# Autodesk Inventor assembly: pcb
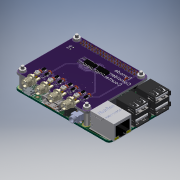
[picture p0: Inventor's stored thumbnail of the model, 180x180]
Saved by Autodesk Inventor 2016 (Build 200138000, 138)
## iProperties
Created: 2016-06-24
Part Number: pcb
Document SubType Name: Assembly
Designer: Jonathan
Author: Jonathan
## Documents named in this file (15)
- C:\Users\Jonathan\Documents\Projects\dynodePiShield\coincidenceCounter\cad\pcb.iam
- C:\Users\Jonathan\Documents\Projects\dynodePiShield\coincidenceCounter\cad\pcb.ipt
- C:\Users\Jonathan\Documents\Projects\dynodePiShield\coincidenceCounter\cad\electronics\SOT23-6.ipt
- C:\Users\Jonathan\Documents\Projects\dynodePiShield\coincidenceCounter\cad\electronics\resistor\chipResistor\chipResistor-0402.ipt
- C:\Users\Jonathan\Documents\Projects\dynodePiShield\coincidenceCounter\cad\electronics\resistor\chipResistor.ipt
- C:\Users\Jonathan\Documents\Projects\dynodePiShield\coincidenceCounter\cad\electronics\PVZ3A\PVZ3A.iam
- C:\Users\Jonathan\Documents\Projects\dynodePiShield\coincidenceCounter\cad\electronics\soic\soic-14-N.ipt
- C:\Users\Jonathan\Documents\Projects\dynodePiShield\coincidenceCounter\cad\electronics\soic\soic.ipt
- C:\Users\Jonathan\Documents\Projects\dynodePiShield\coincidenceCounter\cad\electronics\SMA Female Edge Mount CONSMA003-062.ipt
- C:\Users\Jonathan\Documents\Projects\dynodePiShield\coincidenceCounter\cad\wire.ipt
- C:\Users\Jonathan\Documents\Projects\dynodePiShield\coincidenceCounter\cad\electronics\femaleHeaders\femaleHeaders.iam
- C:\Users\Jonathan\Documents\Projects\dynodePiShield\coincidenceCounter\cad\electronics\raspberrypi_b_+_(assembly).ipt
- C:\Users\Jonathan\Documents\Projects\dynodePiShield\coincidenceCounter\cad\hardware\11mm M2.5 standoff.ipt
- C:\Users\Jonathan\Documents\Projects\dynodePiShield\coincidenceCounter\cad\hardware\M2.5 6mm screw.ipt
- C:\Users\Jonathan\Documents\Projects\dynodePiShield\coincidenceCounter\cad\hardware\M2.5 hex nut.ipt
## Components (54 placed, 12 different names)
1. pcb:1 — Mate:2, Angle:12, Mate:4, Angle:16, Mate:5, Mate:6, Mate:7, Mate:8, Mate:9, Mate:10, Angle:18, Angle:19, Angle:20, Angle:21, Angle:22, Angle:23, Angle:24, Angle:25, Mate:11, Mate:17, Mate:18, Mate:19, Mate:20, Flush:68, Flush:69, Mate:34, Mate:35, Mate:36, Mate:37
2. SOT23-6:1 — Flush:1, Flush:2, Flush:11, Mate:2
3. SOT23-6:2 — Flush:1, Flush:8
4. SOT23-6:3 — Flush:2, Flush:3, Flush:8, Flush:9
5. SOT23-6:4 — Flush:3, Flush:4, Flush:11, Flush:12
6. SOT23-6:5 — Flush:4, Flush:5, Flush:9, Flush:10
7. SOT23-6:6 — Flush:5, Flush:6, Flush:12, Flush:13
8. SOT23-6:7 — Flush:6, Flush:7, Flush:10
9. SOT23-6:8 — Flush:7, Flush:13
10. chipResistor-0402:3 — Flush:28, Flush:46, Mate:9
11. chipResistor-0402:4 — Flush:16, Flush:28, Flush:29, Flush:46
12. chipResistor-0402:7 — Flush:16, Flush:29, Flush:30, Flush:47
13. chipResistor-0402:10 — Flush:30, Flush:47
14. PVZ3A:1 [sub-assembly] — Angle:14, Angle:15, Flush:35, Flush:36, Flush:38, Flush:39, Mate:4
15. PVZ3A:2 [sub-assembly] — Angle:12, Angle:13, Flush:34, Flush:37
16. PVZ3A:3 [sub-assembly] — Angle:13, Angle:14, Flush:34, Flush:35, Flush:37, Flush:38
17. PVZ3A:4 [sub-assembly] — Angle:15, Flush:36, Flush:39
18. soic-14-N:1 — Angle:17, Mate:6
19. soic-14-N:2 — Angle:16, Angle:17, Mate:5
20. SMA Female Edge Mount CONSMA003-062:1 — Flush:42, Flush:45
21. SMA Female Edge Mount CONSMA003-062:2 — Flush:41, Flush:42, Flush:44, Flush:45
22. SMA Female Edge Mount CONSMA003-062:3 — Flush:40, Flush:41, Flush:43, Flush:44
23. SMA Female Edge Mount CONSMA003-062:4 — Flush:40, Flush:43, Mate:7, Mate:8
24. chipResistor-0402:11
25. chipResistor-0402:12
26. chipResistor-0402:13
27. chipResistor-0402:14
28. chipResistor-0402:15
29. chipResistor-0402:16
30. chipResistor-0402:17
31. chipResistor-0402:18
32. wire:1 — Flush:60, Flush:61, Angle:18
33. wire:2 — Flush:60, Flush:65, Mate:10, Angle:19
34. wire:3 — Flush:61, Flush:62, Angle:20
35. wire:4 — Flush:65, Flush:66, Angle:21
36. wire:5 — Flush:62, Flush:63, Angle:22
37. wire:6 — Flush:66, Flush:67, Angle:23
38. wire:7 — Flush:63, Flush:64, Angle:24
39. wire:8 — Flush:67, Angle:25
40. wire:9 — Flush:64
41. femaleHeaders:1 [sub-assembly] — Mate:11, Mate:12
42. raspberrypi_b_+_(assembly):1 — Mate:12, Mate:13, Mate:14, Mate:15, Mate:16, Angle:26, Angle:27, Mate:21, Mate:22, Mate:23, Mate:24, Flush:68, Flush:69, Mate:25, Mate:26, Mate:27, Mate:28
43. 11mm M2.5 standoff:1 — Mate:16, Mate:20, Angle:29, Angle:32, Mate:32, Angle:37
44. 11mm M2.5 standoff:2 — Mate:15, Mate:18, Angle:28, Angle:30, Mate:31, Angle:34
45. 11mm M2.5 standoff:3 — Mate:14, Mate:19, Angle:27, Angle:29, Mate:29, Angle:36
46. 11mm M2.5 standoff:4 — Mate:13, Mate:17, Angle:26, Angle:28, Angle:31, Mate:33, Angle:35
47. M2.5 6mm screw:1 — Mate:21, Mate:28, Angle:30
48. M2.5 6mm screw:2 — Mate:22, Mate:25, Angle:31
49. M2.5 6mm screw:3 — Mate:23, Mate:27, Angle:32, Angle:33
50. M2.5 6mm screw:4 — Mate:24, Mate:26, Angle:33
51. M2.5 hex nut:1 — Mate:33, Mate:34, Angle:35
52. M2.5 hex nut:2 — Mate:31, Mate:36, Angle:34
53. M2.5 hex nut:3 — Mate:32, Mate:37, Angle:37
54. M2.5 hex nut:4 — Mate:29, Mate:35, Angle:36
## Relationships (113: Flush 53, Mate 34, Angle 26)
- Flush:1: SOT23-6:1 ↔ SOT23-6:2
- Flush:2: SOT23-6:1 ↔ SOT23-6:3
- Flush:3: SOT23-6:3 ↔ SOT23-6:4
- Flush:4: SOT23-6:4 ↔ SOT23-6:5
- Flush:5: SOT23-6:5 ↔ SOT23-6:6
- Flush:6: SOT23-6:6 ↔ SOT23-6:7
- Flush:7: SOT23-6:7 ↔ SOT23-6:8
- Flush:8: SOT23-6:2 ↔ SOT23-6:3
- Flush:9: SOT23-6:3 ↔ SOT23-6:5
- Flush:10: SOT23-6:5 ↔ SOT23-6:7
- Flush:11: SOT23-6:1 ↔ SOT23-6:4
- Flush:12: SOT23-6:4 ↔ SOT23-6:6
- Flush:13: SOT23-6:6 ↔ SOT23-6:8
- Mate:2: pcb:1 ↔ SOT23-6:1
- Flush:16: chipResistor-0402:4 ↔ chipResistor-0402:7
- Flush:28: chipResistor-0402:3 ↔ chipResistor-0402:4
- Flush:29: chipResistor-0402:4 ↔ chipResistor-0402:7
- Flush:30: chipResistor-0402:7 ↔ chipResistor-0402:10
- Angle:12 (0 deg): pcb:1 ↔ PVZ3A:2
- Angle:13 (0 deg): PVZ3A:2 ↔ PVZ3A:3
- Angle:14 (0 deg): PVZ3A:1 ↔ PVZ3A:3
- Angle:15 (0 deg): PVZ3A:1 ↔ PVZ3A:4
- Flush:34: PVZ3A:2 ↔ PVZ3A:3
- Flush:35: PVZ3A:1 ↔ PVZ3A:3
- Flush:36: PVZ3A:1 ↔ PVZ3A:4
- Flush:37: PVZ3A:2 ↔ PVZ3A:3
- Flush:38: PVZ3A:1 ↔ PVZ3A:3
- Flush:39: PVZ3A:1 ↔ PVZ3A:4
- Mate:4: pcb:1 ↔ PVZ3A:1
- Angle:16 (0 deg): pcb:1 ↔ soic-14-N:2
- Angle:17 (0 deg): soic-14-N:1 ↔ soic-14-N:2
- Mate:5: pcb:1 ↔ soic-14-N:2
- Mate:6: pcb:1 ↔ soic-14-N:1
- Flush:40: SMA Female Edge Mount CONSMA003-062:3 ↔ SMA Female Edge Mount CONSMA003-062:4
- Flush:41: SMA Female Edge Mount CONSMA003-062:2 ↔ SMA Female Edge Mount CONSMA003-062:3
- Flush:42: SMA Female Edge Mount CONSMA003-062:1 ↔ SMA Female Edge Mount CONSMA003-062:2
- Flush:43: SMA Female Edge Mount CONSMA003-062:3 ↔ SMA Female Edge Mount CONSMA003-062:4
- Flush:44: SMA Female Edge Mount CONSMA003-062:2 ↔ SMA Female Edge Mount CONSMA003-062:3
- Flush:45: SMA Female Edge Mount CONSMA003-062:1 ↔ SMA Female Edge Mount CONSMA003-062:2
- Mate:7: pcb:1 ↔ SMA Female Edge Mount CONSMA003-062:4
- Mate:8: pcb:1 ↔ SMA Female Edge Mount CONSMA003-062:4
- Flush:46: chipResistor-0402:3 ↔ chipResistor-0402:4
- Flush:47: chipResistor-0402:7 ↔ chipResistor-0402:10
- Mate:9: pcb:1 ↔ chipResistor-0402:3
- [Flush]: chipResistor-0402:12 ↔ chipResistor-0402:13
- [Flush]: chipResistor-0402:11 ↔ chipResistor-0402:12
- [Flush]: chipResistor-0402:12 ↔ chipResistor-0402:13
- [Flush]: chipResistor-0402:13 ↔ chipResistor-0402:14
- [Flush]: chipResistor-0402:11 ↔ chipResistor-0402:12
- [Flush]: chipResistor-0402:13 ↔ chipResistor-0402:14
- [Flush]: chipResistor-0402:16 ↔ chipResistor-0402:17
- [Flush]: chipResistor-0402:15 ↔ chipResistor-0402:16
- [Flush]: chipResistor-0402:16 ↔ chipResistor-0402:17
- [Flush]: chipResistor-0402:17 ↔ chipResistor-0402:18
- [Flush]: chipResistor-0402:15 ↔ chipResistor-0402:16
- [Flush]: chipResistor-0402:17 ↔ chipResistor-0402:18
- Flush:60: wire:1 ↔ wire:2
- Flush:61: wire:1 ↔ wire:3
- Flush:62: wire:3 ↔ wire:5
- Flush:63: wire:5 ↔ wire:7
- Flush:64: wire:7 ↔ wire:9
- Flush:65: wire:2 ↔ wire:4
- Flush:66: wire:4 ↔ wire:6
- Flush:67: wire:6 ↔ wire:8
- Mate:10: pcb:1 ↔ wire:2
- Angle:18 (0 deg): pcb:1 ↔ wire:1
- Angle:19 (0 deg): pcb:1 ↔ wire:2
- Angle:20 (0 deg): pcb:1 ↔ wire:3
- Angle:21 (0 deg): pcb:1 ↔ wire:4
- Angle:22 (0 deg): pcb:1 ↔ wire:5
- Angle:23 (0 deg): pcb:1 ↔ wire:6
- Angle:24 (0 deg): pcb:1 ↔ wire:7
- Angle:25 (0 deg): pcb:1 ↔ wire:8
- Mate:11: pcb:1 ↔ femaleHeaders:1
- Mate:12: femaleHeaders:1 ↔ raspberrypi_b_+_(assembly):1
- Mate:13: raspberrypi_b_+_(assembly):1 ↔ 11mm M2.5 standoff:4
- Mate:14: raspberrypi_b_+_(assembly):1 ↔ 11mm M2.5 standoff:3
- Mate:15: raspberrypi_b_+_(assembly):1 ↔ 11mm M2.5 standoff:2
- Mate:16: raspberrypi_b_+_(assembly):1 ↔ 11mm M2.5 standoff:1
- Mate:17: pcb:1 ↔ 11mm M2.5 standoff:4
- Mate:18: pcb:1 ↔ 11mm M2.5 standoff:2
- Mate:19: pcb:1 ↔ 11mm M2.5 standoff:3
- Mate:20: pcb:1 ↔ 11mm M2.5 standoff:1
- Angle:26 (0 deg): raspberrypi_b_+_(assembly):1 ↔ 11mm M2.5 standoff:4
- Angle:27 (0 deg): raspberrypi_b_+_(assembly):1 ↔ 11mm M2.5 standoff:3
- Angle:28 (0 deg): 11mm M2.5 standoff:2 ↔ 11mm M2.5 standoff:4
- Angle:29 (0 deg): 11mm M2.5 standoff:1 ↔ 11mm M2.5 standoff:3
- Mate:21: raspberrypi_b_+_(assembly):1 ↔ M2.5 6mm screw:1
- Mate:22: raspberrypi_b_+_(assembly):1 ↔ M2.5 6mm screw:2
- Mate:23: raspberrypi_b_+_(assembly):1 ↔ M2.5 6mm screw:3
- Mate:24: raspberrypi_b_+_(assembly):1 ↔ M2.5 6mm screw:4
- Flush:68: pcb:1 ↔ raspberrypi_b_+_(assembly):1
- Flush:69: pcb:1 ↔ raspberrypi_b_+_(assembly):1
- Mate:25: raspberrypi_b_+_(assembly):1 ↔ M2.5 6mm screw:2
- Mate:26: raspberrypi_b_+_(assembly):1 ↔ M2.5 6mm screw:4
- Mate:27: raspberrypi_b_+_(assembly):1 ↔ M2.5 6mm screw:3
- Mate:28: raspberrypi_b_+_(assembly):1 ↔ M2.5 6mm screw:1
- Angle:30 (0 deg): 11mm M2.5 standoff:2 ↔ M2.5 6mm screw:1
- Angle:31 (0 deg): 11mm M2.5 standoff:4 ↔ M2.5 6mm screw:2
- Angle:32 (0 deg): 11mm M2.5 standoff:1 ↔ M2.5 6mm screw:3
- Angle:33 (0 deg): M2.5 6mm screw:3 ↔ M2.5 6mm screw:4
- Mate:29: 11mm M2.5 standoff:3 ↔ M2.5 hex nut:4
- Mate:31: 11mm M2.5 standoff:2 ↔ M2.5 hex nut:2
- Mate:32: 11mm M2.5 standoff:1 ↔ M2.5 hex nut:3
- Mate:33: 11mm M2.5 standoff:4 ↔ M2.5 hex nut:1
- Mate:34: pcb:1 ↔ M2.5 hex nut:1
- Mate:35: pcb:1 ↔ M2.5 hex nut:4
- Mate:36: pcb:1 ↔ M2.5 hex nut:2
- Mate:37: pcb:1 ↔ M2.5 hex nut:3
- Angle:34 (0 deg): 11mm M2.5 standoff:2 ↔ M2.5 hex nut:2
- Angle:35 (0 deg): 11mm M2.5 standoff:4 ↔ M2.5 hex nut:1
- Angle:36 (0 deg): 11mm M2.5 standoff:3 ↔ M2.5 hex nut:4
- Angle:37 (0 deg): 11mm M2.5 standoff:1 ↔ M2.5 hex nut:3
## Named parameters: d93_d90 = 0 mm, d94_d91 = 0 mm, d95_d40 = 0 mm, d96_d53 = 0 mm, d97_d54 = 0 mm, d98_d55 = 0 mm, d99_d90 = 0 mm, d100_d91 = 0 mm, d101_d40 = 0 mm, d102_d53 = 0 mm, d103_d54 = 0 mm, d104_d55 = 0 mm
